# Autodesk Inventor assembly: Assembly1
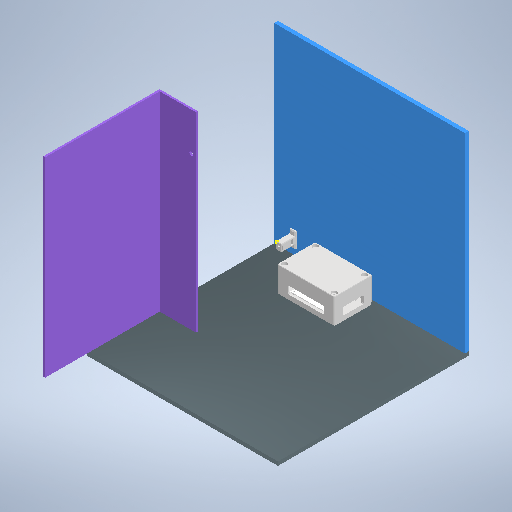
[picture p0: Inventor's stored thumbnail of the model, 512x512]
Saved by Autodesk Inventor 2025.3 (Build 293356000, 356)
## iProperties
Created: 2025-11-14
Part Number: Assembly1
Document SubType Name: Assembly
Designer: woyao
Author: woyao
## Documents named in this file (6)
- D:\Sabi\gogogo\KIT\Hiwi\WBK_Mikrocontroller\Lasersensor+MQTT\Sensor\sensor_demo_2\Assembly1.iam
- D:\Sabi\gogogo\KIT\Hiwi\WBK_Mikrocontroller\Lasersensor+MQTT\Sensor\sensor_demo_2\wall.ipt
- D:\Sabi\gogogo\KIT\Hiwi\WBK_Mikrocontroller\Lasersensor+MQTT\Sensor\sensor_demo_2\door.ipt
- D:\Sabi\gogogo\KIT\Hiwi\WBK_Mikrocontroller\Lasersensor+MQTT\Sensor\sensor_demo_2\VL53L0X_assembly_1.iam
- D:\Sabi\gogogo\KIT\Hiwi\WBK_Mikrocontroller\Lasersensor+MQTT\Sensor\sensor_demo_2\floor.ipt
- D:\Sabi\gogogo\KIT\Hiwi\WBK_Mikrocontroller\Lasersensor+MQTT\Sensor\sensor_demo_2\PCB_Case_Assembly1.iam
## Components (5 placed, 5 different names)
1. wall:1 — Flush:1, Flush:2, Mate:1, Mate:6, Mate:7, Flush:3, Mate:8, Mate:9, Mate:11
2. door:1 — Flush:1, Flush:2, Mate:6
3. VL53L0X_assembly_1:1 [sub-assembly] — Mate:9
4. floor:1 — Mate:7, Flush:3, Mate:8, Mate:12
5. PCB_Case_Assembly1:1 [sub-assembly] — Mate:11, Mate:12
## Relationships (10: Mate 7, Flush 3)
- Flush:1: wall:1 ↔ door:1
- Flush:2: wall:1 ↔ door:1
- Mate:1: wall:1
- Mate:6: wall:1 ↔ door:1
- Mate:7: wall:1 ↔ floor:1
- Flush:3: wall:1 ↔ floor:1
- Mate:8: wall:1 ↔ floor:1
- Mate:9: wall:1 ↔ VL53L0X_assembly_1:1
- Mate:11 (10 mm): wall:1 ↔ PCB_Case_Assembly1:1
- Mate:12: floor:1 ↔ PCB_Case_Assembly1:1
